# Autodesk Inventor assembly: PumpeV6
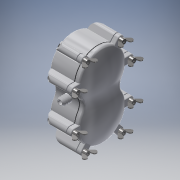
[picture p0: Inventor's stored thumbnail of the model, 180x180]
Saved by Autodesk Inventor 2017 (Build 210142000, 142)
## iProperties
Created: 2019-05-24
Part Number: PumpeV6
Document SubType Name: Assembly
Designer: Ole Simmering
Author: Ole Simmering
## Documents named in this file (8)
- C:\Users\Ole Simmering\Documents\3d modelling fun\HA4-Zahnradpumpe\PumpeV6.iam
- C:\Users\Ole Simmering\Documents\3d modelling fun\HA4-Zahnradpumpe\Gehaeuse_V6.ipt
- C:\Users\Ole Simmering\Documents\3d modelling fun\HA4-Zahnradpumpe\Zahnrad95x50.ipt
- C:\Users\Ole Simmering\Documents\Inventor\Content Center Files\R2017\en-US\ISO 4014(2)\ISO 4014 - M6 x 60 - ISO.ipt
- C:\Users\Ole Simmering\Documents\3d modelling fun\HA4-Zahnradpumpe\Dichtung.ipt
- C:\Users\Ole Simmering\Documents\3d modelling fun\HA4-Zahnradpumpe\Deckel.ipt
- C:\Users\Ole Simmering\Documents\Inventor\Content Center Files\R2017\en-US\Bearing GB_T 292-2007\Rolling bearing B708 C GB_T 292-2007.ipt
- C:\Users\Ole Simmering\Documents\Inventor\Content Center Files\R2017\en-US\DIN 315\DIN 315 - M6.ipt
## Components (25 placed, 7 different names)
1. Dichtung:1 — Mate:7, Mate:8, Mate:9
2. Gehaeuse_V6:1 — Insert:3, Mate:1, Mate:2, Insert:4, Insert:5, Insert:6, Insert:7, Insert:8, Insert:9, Insert:10, Insert:11, Angle:1, Angle:2, Angle:3, Angle:4, Angle:5, Angle:6, Angle:7, Angle:8, Angle:9, Mate:7, Mate:8
3. Zahnrad95x50:1 — Mate:3, Mate:4
4. Zahnrad95x50:2 — Mate:5, Mate:6
5. Deckel:1 — Mate:9, Mate:10, Mate:11, Mate:28, Mate:29, Mate:30, Mate:31, Insert:12, Insert:13, Insert:14, Insert:15, Insert:16, Insert:17, Insert:18, Insert:19
6. Bearing GB/T 292-2007 Type IN - withdrawn B708 C:1 — Insert:3, Mate:3, Mate:4
7. Bearing GB/T 292-2007 Type IN - withdrawn B708 C:2 — Mate:1, Mate:2, Mate:5, Mate:6
8. Bearing GB/T 292-2007 Type IN - withdrawn B708 C:3 — Mate:28, Mate:29
9. Bearing GB/T 292-2007 Type IN - withdrawn B708 C:4 — Mate:30, Mate:31
10. DIN 315 M6:5 — Insert:12
11. DIN 315 M6:6 — Insert:13
12. DIN 315 M6:7 — Insert:14
13. DIN 315 M6:8 — Insert:15
14. DIN 315 M6:9 — Insert:16
15. DIN 315 M6:10 — Insert:17
16. DIN 315 M6:11 — Insert:18
17. DIN 315 M6:12 — Insert:19
18. ISO 4014 M6 x 60:1 — Insert:10, Angle:2
19. ISO 4014 M6 x 60:2 — Insert:11, Angle:5
20. ISO 4014 M6 x 60:3 — Insert:9, Angle:3
21. ISO 4014 M6 x 60:4 — Insert:4, Angle:4, Mate:11
22. ISO 4014 M6 x 60:5 — Insert:5, Angle:1, Angle:6
23. ISO 4014 M6 x 60:6 — Insert:6, Angle:9
24. ISO 4014 M6 x 60:7 — Insert:7, Angle:8, Mate:10
25. ISO 4014 M6 x 60:8 — Insert:8, Angle:7
## Relationships (41: Insert 17, Mate 15, Angle 9)
- Insert:3: Gehaeuse_V6:1 ↔ Bearing GB/T 292-2007 Type IN - withdrawn B708 C:1
- Mate:1: Gehaeuse_V6:1 ↔ Bearing GB/T 292-2007 Type IN - withdrawn B708 C:2
- Mate:2: Gehaeuse_V6:1 ↔ Bearing GB/T 292-2007 Type IN - withdrawn B708 C:2
- Mate:3: Zahnrad95x50:1 ↔ Bearing GB/T 292-2007 Type IN - withdrawn B708 C:1
- Mate:4: Zahnrad95x50:1 ↔ Bearing GB/T 292-2007 Type IN - withdrawn B708 C:1
- Mate:5: Zahnrad95x50:2 ↔ Bearing GB/T 292-2007 Type IN - withdrawn B708 C:2
- Mate:6: Zahnrad95x50:2 ↔ Bearing GB/T 292-2007 Type IN - withdrawn B708 C:2
- Insert:4: Gehaeuse_V6:1 ↔ ISO 4014 M6 x 60:4
- Insert:5: Gehaeuse_V6:1 ↔ ISO 4014 M6 x 60:5
- Insert:6: Gehaeuse_V6:1 ↔ ISO 4014 M6 x 60:6
- Insert:7: Gehaeuse_V6:1 ↔ ISO 4014 M6 x 60:7
- Insert:8: Gehaeuse_V6:1 ↔ ISO 4014 M6 x 60:8
- Insert:9: Gehaeuse_V6:1 ↔ ISO 4014 M6 x 60:3
- Insert:10: Gehaeuse_V6:1 ↔ ISO 4014 M6 x 60:1
- Insert:11: Gehaeuse_V6:1 ↔ ISO 4014 M6 x 60:2
- Angle:1 (0 deg): Gehaeuse_V6:1 ↔ ISO 4014 M6 x 60:5
- Angle:2 (0 deg): Gehaeuse_V6:1 ↔ ISO 4014 M6 x 60:1
- Angle:3 (0 deg): Gehaeuse_V6:1 ↔ ISO 4014 M6 x 60:3
- Angle:4 (0 deg): Gehaeuse_V6:1 ↔ ISO 4014 M6 x 60:4
- Angle:5 (0 deg): Gehaeuse_V6:1 ↔ ISO 4014 M6 x 60:2
- Angle:6 (0 deg): Gehaeuse_V6:1 ↔ ISO 4014 M6 x 60:5
- Angle:7 (0 deg): Gehaeuse_V6:1 ↔ ISO 4014 M6 x 60:8
- Angle:8 (0 deg): Gehaeuse_V6:1 ↔ ISO 4014 M6 x 60:7
- Angle:9 (0 deg): Gehaeuse_V6:1 ↔ ISO 4014 M6 x 60:6
- Mate:7: Dichtung:1 ↔ Gehaeuse_V6:1
- Mate:8: Dichtung:1 ↔ Gehaeuse_V6:1
- Mate:9: Dichtung:1 ↔ Deckel:1
- Mate:10: Deckel:1 ↔ ISO 4014 M6 x 60:7
- Mate:11: Deckel:1 ↔ ISO 4014 M6 x 60:4
- Mate:28: Deckel:1 ↔ Bearing GB/T 292-2007 Type IN - withdrawn B708 C:3
- Mate:29: Deckel:1 ↔ Bearing GB/T 292-2007 Type IN - withdrawn B708 C:3
- Mate:30: Deckel:1 ↔ Bearing GB/T 292-2007 Type IN - withdrawn B708 C:4
- Mate:31: Deckel:1 ↔ Bearing GB/T 292-2007 Type IN - withdrawn B708 C:4
- Insert:12: Deckel:1 ↔ DIN 315 M6:5
- Insert:13: Deckel:1 ↔ DIN 315 M6:6
- Insert:14: Deckel:1 ↔ DIN 315 M6:7
- Insert:15: Deckel:1 ↔ DIN 315 M6:8
- Insert:16: Deckel:1 ↔ DIN 315 M6:9
- Insert:17: Deckel:1 ↔ DIN 315 M6:10
- Insert:18: Deckel:1 ↔ DIN 315 M6:11
- Insert:19: Deckel:1 ↔ DIN 315 M6:12
